# Autodesk Inventor assembly: Motor with Screw Generator
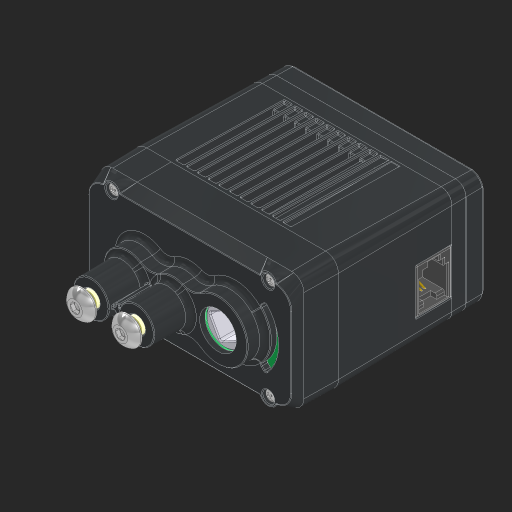
[picture p0: Inventor's stored thumbnail of the model, 512x512]
Saved by Autodesk Inventor 2023 (Build 270158000, 158)
## iProperties
Created: 2021-07-20
Part Number: Motor with Screw Generator
Document SubType Name: Assembly
Designer: yuany
Author: yuany
## Documents named in this file (4)
- C:\Users\ylu12\Documents\GitHub\VEX-CAD-Inventor\Electronics\Motors with Screws\Motor with Screw Generator.iam
- C:\Users\ylu12\Documents\GitHub\VEX-CAD-Inventor\Electronics\V5 Motor.ipt
- C:\Users\ylu12\Documents\GitHub\VEX-CAD-Inventor\Structure\Hardware\Screw Steel - Hex\SScrew Hex Threaded .500.ipt
- C:\Users\ylu12\Documents\GitHub\VEX-CAD-Inventor\Structure\Hardware\Screw Steel - Hex.ipt
## Components (3 placed, 2 different names)
1. V5 Motor:1
2. SScrew Hex Threaded .500:1
3. SScrew Hex Threaded .500:2
## Relationships (2: Insert 2)
- [Insert] (1.5875 mm): V5 Motor:1 ↔ SScrew Hex Threaded .500:1
- [Insert] (1.5875 mm): V5 Motor:1 ↔ SScrew Hex Threaded .500:2
## Named parameters: Thick = 1.5875 mm
